# Autodesk Inventor assembly: Leg_Right_v1
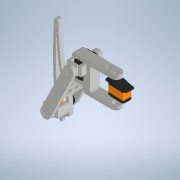
[picture p0: Inventor's stored thumbnail of the model, 180x180]
Saved by Autodesk Inventor 2020.3 (Build 243373000, 373)
## iProperties
Created: 2021-03-06
Part Number: Leg_Right_v1
Document SubType Name: Assembly
Designer: sanyi
Author: sanyi
## Documents named in this file (6)
- C:\Users\sanyi\OneDrive\Dokumentumok\Inventor\Quadropod\Leg_Right_v1.iam
- C:\Users\sanyi\OneDrive\Dokumentumok\Inventor\Quadropod\LegEnd_Right_v1.ipt
- C:\Users\sanyi\OneDrive\Dokumentumok\Inventor\Quadropod\LegMiddle_Final_1.ipt
- C:\Users\sanyi\OneDrive\Dokumentumok\Inventor\Quadropod\LegPin_v1.ipt
- C:\Users\sanyi\OneDrive\Dokumentumok\Inventor\Quadropod\LegStart_v1.ipt
- C:\Users\sanyi\OneDrive\Dokumentumok\Inventor\Quadropod\SH-0257MG.ipt
## Components (8 placed, 5 different names)
1. LegStart_v1:1 — Mate:4, Angle:1, Mate:6, Mate:7, Mate:8, Insert:8, Insert:9, Insert:10, Mate:10, Mate:11, Flush:1
2. LegEnd_Right_v1:1 — Mate:2, Mate:5, Insert:7, Angle:2, Mate:9, Insert:11, Insert:12
3. LegMiddle_Final_1:1 — Insert:6, Insert:13
4. LegPin_v1:1 — Mate:8, Insert:8, Insert:9, Insert:13
5. LegPin_v1:2 — Mate:2, Insert:6, Mate:9, Insert:11, Insert:12
6. SH-0257MG:1 — Mate:4, Angle:1, Insert:10
7. SH-0257MG:2 — Mate:6, Mate:7
8. SH-0257MG:3 — Mate:5, Insert:7, Angle:2
## Relationships (20: Mate 9, Insert 8, Angle 2, Flush 1)
- Mate:2: LegEnd_Right_v1:1 ↔ LegPin_v1:2
- Mate:4: LegStart_v1:1 ↔ SH-0257MG:1
- Angle:1 (0 deg): LegStart_v1:1 ↔ SH-0257MG:1
- Insert:6 (0.2 mm): LegMiddle_Final_1:1 ↔ LegPin_v1:2
- Mate:5: LegEnd_Right_v1:1 ↔ SH-0257MG:3
- Insert:7: LegEnd_Right_v1:1 ↔ SH-0257MG:3
- Angle:2 (0 deg): LegEnd_Right_v1:1 ↔ SH-0257MG:3
- Mate:6: LegStart_v1:1 ↔ SH-0257MG:2
- Mate:7: LegStart_v1:1 ↔ SH-0257MG:2
- Mate:8: LegStart_v1:1 ↔ LegPin_v1:1
- Insert:8: LegStart_v1:1 ↔ LegPin_v1:1
- Insert:9: LegStart_v1:1 ↔ LegPin_v1:1
- Insert:10: LegStart_v1:1 ↔ SH-0257MG:1
- Mate:9: LegEnd_Right_v1:1 ↔ LegPin_v1:2
- Insert:11: LegEnd_Right_v1:1 ↔ LegPin_v1:2
- Insert:12: LegEnd_Right_v1:1 ↔ LegPin_v1:2
- Mate:10: LegStart_v1:1
- Mate:11: LegStart_v1:1
- Flush:1: LegStart_v1:1
- Insert:13 (0.2 mm): LegMiddle_Final_1:1 ↔ LegPin_v1:1
